# Autodesk Inventor assembly: holder_wheel_pair
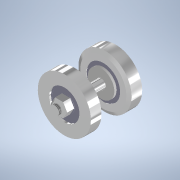
[picture p0: Inventor's stored thumbnail of the model, 180x180]
Saved by Autodesk Inventor 2020.3 (Build 243373000, 373)
## iProperties
Created: 2021-03-25
Part Number: holder_wheel_pair
Document SubType Name: Assembly
Designer: patry
Mass: 73.5609 g
Surface Area: 155.822 cm^2
Volume: 27.2448 cm^3
Density: 2.7 g/cm^3
Author: patry
## Documents named in this file (6)
- C:\Users\patry\Desktop\Semestr 7\Inzynierka\Projekt inventor\Ariadna_inzynierka\Workspaces\Obszar roboczy\Obszar roboczy\Naped\Kola\holder_wheel_pair.iam
- C:\Users\patry\Desktop\Semestr 7\Inzynierka\Projekt inventor\Ariadna_inzynierka\Workspaces\Obszar roboczy\Obszar roboczy\Naped\Sruby\M5_nut_5mm.ipt
- C:\Users\patry\Desktop\Semestr 7\Inzynierka\Projekt inventor\Ariadna_inzynierka\Workspaces\Obszar roboczy\Obszar roboczy\Naped\Sruby\M5_40_shaft.ipt
- M5_shaft.ipt
- C:\Users\patry\Desktop\Semestr 7\Inzynierka\Projekt inventor\Ariadna_inzynierka\Workspaces\Obszar roboczy\Obszar roboczy\Naped\Kola\single_wheel_dummie.iam
- C:\Users\patry\Desktop\Semestr 7\Inzynierka\Projekt inventor\Ariadna_inzynierka\Workspaces\Obszar roboczy\Obszar roboczy\Naped\Sruby\M5_pad.ipt
## Components (7 placed, 4 different names)
1. M5_nut_5mm:1 — Zestawiające:17, Zestawiające:18, Zestawiające:20
2. M5_shaft:1 — Zestawiające:16, Zestawiające:18, Równoległe:1, Zestawiające:19, Zestawiające:21, Zestawiające:23, Zestawiające:25
3. M5_nut_5mm:5 — Zestawiające:16, Zestawiające:17, Równoległe:1, Zestawiające:22
4. single_wheel_dummie:1 [sub-assembly] — Zestawiające:19, Zestawiające:20, Zestawiające:26
5. single_wheel_dummie:2 [sub-assembly] — Zestawiające:21, Zestawiające:22, Zestawiające:24
6. M5_pad:1 — Zestawiające:23, Zestawiające:24
7. M5_pad:2 — Zestawiające:25, Zestawiające:26
## Relationships (12: Mate 11, Flush 1)
- Zestawiające:16 [Mate]: M5_shaft:1 ↔ M5_nut_5mm:5
- Zestawiające:17 [Mate] (27 mm): M5_nut_5mm:1 ↔ M5_nut_5mm:5
- Zestawiające:18 [Mate]: M5_nut_5mm:1 ↔ M5_shaft:1
- Równoległe:1 [Flush] (1.5 mm): M5_shaft:1 ↔ M5_nut_5mm:5
- Zestawiające:19 [Mate]: M5_shaft:1 ↔ single_wheel_dummie:1
- Zestawiające:20 [Mate]: M5_nut_5mm:1 ↔ single_wheel_dummie:1
- Zestawiające:21 [Mate]: M5_shaft:1 ↔ single_wheel_dummie:2
- Zestawiające:22 [Mate]: M5_nut_5mm:5 ↔ single_wheel_dummie:2
- Zestawiające:23 [Mate]: M5_shaft:1 ↔ M5_pad:1
- Zestawiające:24 [Mate]: single_wheel_dummie:2 ↔ M5_pad:1
- Zestawiające:25 [Mate]: M5_shaft:1 ↔ M5_pad:2
- Zestawiające:26 [Mate]: single_wheel_dummie:1 ↔ M5_pad:2
